# Autodesk Inventor assembly: parts_combined_3D_Printer_2_Bumper
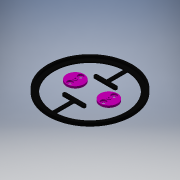
[picture p0: Inventor's stored thumbnail of the model, 180x180]
Saved by Autodesk Inventor 2016 (Build 200138000, 138)
## iProperties
Created: 2016-07-26
Part Number: parts_combined_3D_Printer_2_Bumper
Material: Générique
Document SubType Name: Assembly
Designer: tmonglon
Author: tmonglon
## Documents named in this file (3)
- D:\Inventor\Ahmet\AAA\chassis-nov2016\design\set2_to_print.iam
- D:\Inventor\Ahmet\AAA\chassis-nov2016\design\magnet_holder.ipt
- D:\Inventor\Ahmet\AAA\chassis-nov2016\design\bumper.ipt
## Components (3 placed, 2 different names)
1. magnet_holder:1 — Placage:3, Angle:1, Affleurement:1, Placage:6
2. magnet_holder:2 — Placage:4, Angle:2, Affleurement:1, Placage:7
3. bumper:1 — Placage:1, Placage:2, Angle:1, Angle:2, Placage:5
## Relationships (10: Mate 7, Angle 2, Flush 1)
- Placage:1 [Mate]: bumper:1
- Placage:2 [Mate]: bumper:1
- Placage:3 [Mate]: magnet_holder:1
- Placage:4 [Mate]: magnet_holder:2
- Angle:1 (90 deg): magnet_holder:1 ↔ bumper:1
- Angle:2 (90 deg): magnet_holder:2 ↔ bumper:1
- Placage:5 [Mate]: bumper:1
- Affleurement:1 [Flush]: magnet_holder:1 ↔ magnet_holder:2
- Placage:6 [Mate]: magnet_holder:1
- Placage:7 [Mate]: magnet_holder:2
